# Autodesk Inventor assembly: mcu_board
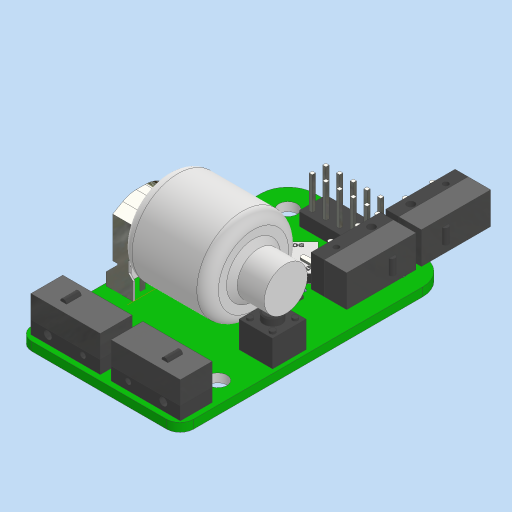
[picture p0: Inventor's stored thumbnail of the model, 512x512]
Saved by Autodesk Inventor 2024 (Build 280153000, 153)
## iProperties
Created: 2025-05-06
Part Number: mcu_board
Document SubType Name: Assembly
Designer: XxPan
Author: XxPan
## iProperties of the stored document CAP_0603.ipt
Created: 2025-05-07
Part Number: product
Material: Generic
Description: STEP AP214
Document SubType Name: Modeling
Designer: XxPan
Density: 1 g/cm^3
Appearance: Default
Title: CAP_CL10_SAM
Revision Number: 1.0first version
## iProperties of the stored document CAP_0402.ipt
Created: 2025-05-06
Part Number: product
Material: Generic
Description: STEP AP214
Document SubType Name: Modeling
Designer: XxPan
Density: 1 g/cm^3
Appearance: Default
Title: CAP_CL05_SAM
Revision Number: 1.0first version
## iProperties of the stored document RES_0402.ipt
Created: 2025-05-06
Part Number: product
Material: Generic
Description: STEP AP214
Document SubType Name: Modeling
Designer: XxPan
Density: 1 g/cm^3
Appearance: Default
Title: RC0402N_YAG
Revision Number: 1.0first version
## iProperties of the stored document CAP_0805.ipt
Created: 2025-05-06
Part Number: product
Material: Generic
Description: STEP AP214
Document SubType Name: Modeling
Designer: XxPan
Density: 1 g/cm^3
Appearance: Default
Title: CAP_CL21_SAM
Revision Number: 1.0first version
## iProperties of the stored document 44PW_ATM.ipt
Created: 2025-05-06
Part Number: product
Material: Generic
Description: STEP AP214
Document SubType Name: Modeling
Designer: XxPan
Density: 1 g/cm^3
Appearance: Default
Title: 44PW_ATM
Revision Number: 1.0first version
## iProperties of the stored document CAP_0201.ipt
Created: 2024-08-04
Part Number: GRM_Auto_Q3_0.6_0.3_0.33_0.15
Material: Generic
Description: STEP AP214
Document SubType Name: Modeling
Designer: XxPan
Density: 1 g/cm^3
Appearance: Default
Sending System: SolidWorks 2021
Preprocessor: SwSTEP 2.0
Title: GRM_Auto_Q3_0.6_0.3_0.33_0.15.STEP
Revision Number: ANY
## Documents named in this file (22)
- C:\Users\XxPan\OneDrive - McMaster University\Mouse\CAD\mcu_board.iam
- **C:\Users\XxPan\OneDrive - McMaster University\Mouse\CAD\mcu_board.iam*LocalDocs*xAaaaaddaAaaaaaaaAaaaajjlXb*44PW_ATM.ipt
- C:\Users\XxPan\OneDrive - McMaster University\Mouse\CAD\6mm_switch.ipt
- C:\Users\XxPan\OneDrive - McMaster University\Mouse\CAD\Kailh_GM_8.0_switch.ipt
- C:\Users\XxPan\OneDrive - McMaster University\Mouse\CAD\TTC_silver_rotary_encoder.ipt
- C:\Users\XxPan\OneDrive - McMaster University\Mouse\CAD\mcu_pcb.ipt
- C:\Users\XxPan\OneDrive - McMaster University\Mouse\CAD\crystal_oscillator.ipt
- **C:\Users\XxPan\OneDrive - McMaster University\Mouse\CAD\mcu_board.iam*LocalDocs*xAaaaqxcaAaaaaaaaAaaaamazQe*CAP_0201.ipt
- **C:\Users\XxPan\OneDrive - McMaster University\Mouse\CAD\mcu_board.iam*LocalDocs*xAaaaaddaAaaaaaaaAaaaajjlDc*CAP_0402.ipt
- **C:\Users\XxPan\OneDrive - McMaster University\Mouse\CAD\mcu_board.iam*LocalDocs*xAaaaaddaAaaaaaaaAaaaajjlEc*CAP_0603.ipt
- **C:\Users\XxPan\OneDrive - McMaster University\Mouse\CAD\mcu_board.iam*LocalDocs*xAaaaaddaAaaaaaaaAaaaajjlFc*CAP_0805.ipt
- **C:\Users\XxPan\OneDrive - McMaster University\Mouse\CAD\mcu_board.iam*LocalDocs*xAaaaaddaAaaaaaaaAaaaajjlGc*RES_0402.ipt
- C:\Users\XxPan\OneDrive - McMaster University\Mouse\CAD\scroll_wheel.ipt
- C:\Users\XxPan\OneDrive - McMaster University\Mouse\CAD\2x5_P2.54mm_male_header.ipt
- C:\Users\XxPan\OneDrive - McMaster University\Mouse\CAD\mcu_label.ipt
- C:\Users\XxPan\OneDrive - McMaster University\Mouse\CAD\R-667842_tactile_switch.ipt
- C:\Users\XxPan\OneDrive - McMaster University\Mouse\CAD_models\ATMEGA32U4_MU\44PW_ATM.step
- C:\Users\XxPan\OneDrive - McMaster University\Mouse\CAD_models\capacitors\CAP_0201.step
- C:\Users\XxPan\OneDrive - McMaster University\Mouse\CAD_models\capacitors\CAP_0402.step
- C:\Users\XxPan\OneDrive - McMaster University\Mouse\CAD_models\capacitors\CAP_0603.step
- C:\Users\XxPan\OneDrive - McMaster University\Mouse\CAD_models\capacitors\CAP_0805.step
- C:\Users\XxPan\OneDrive - McMaster University\Mouse\CAD_models\resistors\RES_0402.step
## Components (22 placed, 15 different names)
1. 44PW_ATM:1 — Mate:1, Flush:6, Mate:23, Flush:7, Angle:1
2. 6mm_switch:1 — Mate:5, Flush:9, Flush:10
3. TTC_silver_rotary_encoder:1 — Mate:4, Flush:11, Insert:1
4. mcu_pcb:1 — Mate:1, Mate:2, Mate:3, Mate:4, Mate:5, Mate:6, Mate:7, Mate:8, Mate:9, Mate:10, Mate:11, Mate:12, Mate:15, Mate:16, Mate:20, Mate:22, Angle:1, Flush:8, Mate:24, Flush:10, Flush:11, Mate:25, Mate:26, Flush:12, Flush:13, Flush:14, Flush:15, Mate:27, Flush:16
5. Kailh_GM_8.0_switch:1 — Mate:2, Mate:18, Flush:3
6. Kailh_GM_8.0_switch:2 — Mate:21, Flush:4, Flush:5, Mate:27
7. Kailh_GM_8.0_switch:3 — Mate:21, Flush:4, Flush:5, Mate:22, Flush:16
8. Kailh_GM_8.0_switch:4 — Mate:3, Mate:18, Flush:3, Flush:8
9. crystal_oscillator:1 — Mate:6, Mate:13, Mate:14, Flush:1, Flush:2
10. CAP_0201:1 — Mate:10, Mate:13, Flush:2
11. CAP_0201:2 — Mate:9, Mate:14, Flush:1
12. CAP_0402:1 — Mate:11
13. CAP_0603:1 — Mate:8
14. CAP_0805:1 — Mate:7
15. RES_0402:1 — Mate:12
16. CAP_0402:2 — Mate:15
17. CAP_0402:3 — Mate:16
18. scroll_wheel:1 — Angle:2, Flush:9, Mate:24, Insert:1
19. 2x5_P2.54mm_male_header:1 — Mate:20
20. mcu_label:1 — Flush:6, Mate:23, Flush:7
21. R-667842_tactile_switch:2 — Mate:26, Flush:14, Flush:15
22. R-667842_tactile_switch:1 — Mate:25, Flush:12, Flush:13
## Relationships (44: Mate 25, Flush 16, Angle 2, Insert 1)
- Mate:1: 44PW_ATM:1 ↔ mcu_pcb:1
- Mate:2: mcu_pcb:1 ↔ Kailh_GM_8.0_switch:1
- Mate:3: mcu_pcb:1 ↔ Kailh_GM_8.0_switch:4
- Mate:4: TTC_silver_rotary_encoder:1 ↔ mcu_pcb:1
- Mate:5: 6mm_switch:1 ↔ mcu_pcb:1
- Mate:6: mcu_pcb:1 ↔ crystal_oscillator:1
- Mate:7: mcu_pcb:1 ↔ CAP_0805:1
- Mate:8: mcu_pcb:1 ↔ CAP_0603:1
- Mate:9: mcu_pcb:1 ↔ CAP_0201:2
- Mate:10: mcu_pcb:1 ↔ CAP_0201:1
- Mate:11: mcu_pcb:1 ↔ CAP_0402:1
- Mate:12: mcu_pcb:1 ↔ RES_0402:1
- Mate:13 (1 mm): crystal_oscillator:1 ↔ CAP_0201:1
- Mate:14 (1 mm): crystal_oscillator:1 ↔ CAP_0201:2
- Flush:1 (-1 mm): crystal_oscillator:1 ↔ CAP_0201:2
- Flush:2 (1 mm): crystal_oscillator:1 ↔ CAP_0201:1
- Mate:15: mcu_pcb:1 ↔ CAP_0402:2
- Mate:16: mcu_pcb:1 ↔ CAP_0402:3
- Mate:18 (2 mm): Kailh_GM_8.0_switch:1 ↔ Kailh_GM_8.0_switch:4
- Flush:3: Kailh_GM_8.0_switch:1 ↔ Kailh_GM_8.0_switch:4
- Mate:20: mcu_pcb:1 ↔ 2x5_P2.54mm_male_header:1
- Mate:21 (1 mm): Kailh_GM_8.0_switch:2 ↔ Kailh_GM_8.0_switch:3
- Flush:4: Kailh_GM_8.0_switch:2 ↔ Kailh_GM_8.0_switch:3
- Flush:5: Kailh_GM_8.0_switch:2 ↔ Kailh_GM_8.0_switch:3
- Mate:22 (8 mm): mcu_pcb:1 ↔ Kailh_GM_8.0_switch:3
- Flush:6: 44PW_ATM:1 ↔ mcu_label:1
- Mate:23: 44PW_ATM:1 ↔ mcu_label:1
- Flush:7: 44PW_ATM:1 ↔ mcu_label:1
- Angle:1 (45 deg): 44PW_ATM:1 ↔ mcu_pcb:1
- Flush:8 (1 mm): mcu_pcb:1 ↔ Kailh_GM_8.0_switch:4
- Angle:2 (0 deg): scroll_wheel:1
- Flush:9: 6mm_switch:1 ↔ scroll_wheel:1
- Mate:24 (-29 mm): mcu_pcb:1 ↔ scroll_wheel:1
- Flush:10 (0.75 mm): 6mm_switch:1 ↔ mcu_pcb:1
- Flush:11 (4.4 mm): TTC_silver_rotary_encoder:1 ↔ mcu_pcb:1
- Mate:25: mcu_pcb:1 ↔ R-667842_tactile_switch:1
- Mate:26: mcu_pcb:1 ↔ R-667842_tactile_switch:2
- Flush:12 (2.8 mm): mcu_pcb:1 ↔ R-667842_tactile_switch:1
- Flush:13 (8.9 mm): mcu_pcb:1 ↔ R-667842_tactile_switch:1
- Flush:14 (1.9 mm): mcu_pcb:1 ↔ R-667842_tactile_switch:2
- Flush:15 (9.8 mm): mcu_pcb:1 ↔ R-667842_tactile_switch:2
- Mate:27 (-2 mm): mcu_pcb:1 ↔ Kailh_GM_8.0_switch:2
- Flush:16 (-3 mm): mcu_pcb:1 ↔ Kailh_GM_8.0_switch:3
- Insert:1 (5.5 mm): TTC_silver_rotary_encoder:1 ↔ scroll_wheel:1
